# Autodesk Inventor assembly: Intake Full Assembly
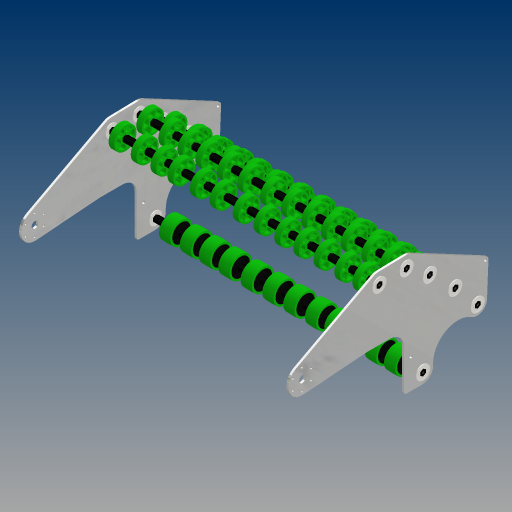
[picture p0: Inventor's stored thumbnail of the model, 512x512]
Saved by Autodesk Inventor 2024.3 (Build 283343000, 343)
## iProperties
Created: 2024-07-29
Part Number: Intake Full Assembly
Document SubType Name: Assembly
Designer: Kenji
Author: Kenji
## Documents named in this file (6)
- C:\Users\Kenji\Documents\GitHub\1622-2024-Summer-CAD-A-Thon\Intake\Intake Full Assembly.iam
- C:\Users\Kenji\Documents\GitHub\1622-2024-Summer-CAD-A-Thon\Intake\Intake Roller Plate.ipt
- C:\Users\Kenji\Documents\GitHub\1622-2024-Summer-CAD-A-Thon\COTS Library\Motion\Bearings\COTS_WCP-0783_1.125ODHexBearing.ipt
- C:\Users\Kenji\Documents\GitHub\1622-2024-Summer-CAD-A-Thon\Intake\Intake HexShaft 1.ipt
- C:\Users\Kenji\Documents\GitHub\1622-2024-Summer-CAD-A-Thon\Intake\am-3462 2IN Molded 500Hex Compliant Wheel REV2.ipt
- C:\Users\Kenji\Documents\GitHub\1622-2024-Summer-CAD-A-Thon\Intake\am-3155 2IN 500Hex Stealth Wheel REV2.iam
## Components (97 placed, 5 different names)
1. Intake Roller Plate:1 — Mate:13, Mate:14, Mate:15, Mate:16, Mate:17, Mate:18, Mate:19, Mate:20, Mate:21, Mate:22, Mate:23, Mate:24
2. Intake Roller Plate:2 — Mate:1, Mate:2, Mate:3, Mate:4, Mate:5, Mate:6, Mate:7, Mate:8, Mate:9, Mate:10, Mate:11, Mate:12
3. COTS_WCP-0783_1.125ODHexBearing:1 — Mate:5, Mate:7, Mate:25, Mate:32, Flush:11
4. COTS_WCP-0783_1.125ODHexBearing:2 — Mate:6, Mate:8, Mate:26, Mate:27, Flush:1
5. COTS_WCP-0783_1.125ODHexBearing:3 — Mate:4, Mate:11, Mate:31, Flush:9
6. COTS_WCP-0783_1.125ODHexBearing:4 — Mate:3, Mate:10, Flush:8
7. COTS_WCP-0783_1.125ODHexBearing:5 — Mate:1, Mate:9, Flush:4
8. COTS_WCP-0783_1.125ODHexBearing:6 — Mate:2, Mate:12, Flush:6
9. COTS_WCP-0783_1.125ODHexBearing:7 — Mate:17, Mate:24, Flush:10
10. COTS_WCP-0783_1.125ODHexBearing:8 — Mate:16, Mate:22, Mate:30, Flush:7
11. COTS_WCP-0783_1.125ODHexBearing:9 — Mate:15, Mate:21, Mate:29, Flush:5
12. COTS_WCP-0783_1.125ODHexBearing:10 — Mate:18, Mate:23, Mate:25, Flush:12
13. COTS_WCP-0783_1.125ODHexBearing:11 — Mate:13, Mate:19, Mate:26, Flush:2
14. COTS_WCP-0783_1.125ODHexBearing:12 — Mate:14, Mate:20, Mate:28, Flush:3, Mate:33, Mate:36, Mate:37, Mate:38, Mate:39, Mate:40
15. Intake HexShaft 1:1 — Mate:31, Flush:9, Flush:10, Mate:73, Mate:74, Mate:75, Mate:76, Mate:77, Mate:78, Mate:79, Mate:80, Mate:81, Mate:82, Mate:83, Mate:84, Mate:85
16. Intake HexShaft 1:2 — Mate:32, Flush:11, Flush:12, Mate:86, Mate:87, Mate:88, Mate:89, Mate:90, Mate:91, Mate:92, Mate:93, Mate:94, Mate:95, Mate:96, Mate:97, Mate:98
17. Intake HexShaft 1:3 — Mate:30, Flush:7, Flush:8, Mate:60, Mate:61, Mate:62, Mate:63, Mate:64, Mate:65, Mate:66, Mate:67, Mate:68, Mate:69, Mate:70, Mate:71, Mate:72
18. Intake HexShaft 1:4 — Mate:29, Flush:5, Flush:6, Mate:47, Mate:48, Mate:49, Mate:50, Mate:51, Mate:52, Mate:53, Mate:54, Mate:55, Mate:56, Mate:57, Mate:58, Mate:59
19. Intake HexShaft 1:5 — Mate:28, Flush:3, Flush:4, Mate:34, Mate:35, Mate:41, Mate:42, Mate:43, Mate:44, Mate:45
20. Intake HexShaft 1:6 — Mate:27, Flush:1, Flush:2, Mate:99, Mate:100, Mate:101, Mate:102, Mate:103, Mate:104, Mate:105, Mate:106, Mate:107, Mate:108, Mate:109, Mate:110
21. am-3462 2IN Molded 500Hex Compliant Wheel REV2:1 — Mate:45
22. am-3462 2IN Molded 500Hex Compliant Wheel REV2:2 — Mate:50
23. am-3462 2IN Molded 500Hex Compliant Wheel REV2:3 — Mate:51
24. am-3462 2IN Molded 500Hex Compliant Wheel REV2:4 — Mate:44
25. am-3462 2IN Molded 500Hex Compliant Wheel REV2:5 — Mate:40
26. am-3462 2IN Molded 500Hex Compliant Wheel REV2:6 — Mate:39
27. am-3462 2IN Molded 500Hex Compliant Wheel REV2:7 — Mate:42
28. am-3462 2IN Molded 500Hex Compliant Wheel REV2:8 — Mate:48
29. am-3462 2IN Molded 500Hex Compliant Wheel REV2:9 — Mate:52
30. am-3462 2IN Molded 500Hex Compliant Wheel REV2:10 — Mate:56
31. am-3462 2IN Molded 500Hex Compliant Wheel REV2:11 — Mate:55
32. am-3462 2IN Molded 500Hex Compliant Wheel REV2:12 — Mate:54
33. am-3462 2IN Molded 500Hex Compliant Wheel REV2:13 — Mate:53
34. am-3462 2IN Molded 500Hex Compliant Wheel REV2:14 — Mate:43
35. am-3462 2IN Molded 500Hex Compliant Wheel REV2:15 — Mate:41
36. am-3462 2IN Molded 500Hex Compliant Wheel REV2:16 — Mate:35
37. am-3462 2IN Molded 500Hex Compliant Wheel REV2:17 — Mate:37
38. am-3462 2IN Molded 500Hex Compliant Wheel REV2:19 — Mate:49
39. am-3462 2IN Molded 500Hex Compliant Wheel REV2:20 — Mate:47
40. am-3462 2IN Molded 500Hex Compliant Wheel REV2:21 — Mate:38
41. am-3462 2IN Molded 500Hex Compliant Wheel REV2:22 — Mate:36
42. am-3462 2IN Molded 500Hex Compliant Wheel REV2:23 — Mate:34
43. am-3462 2IN Molded 500Hex Compliant Wheel REV2:24 — Mate:33
44. am-3462 2IN Molded 500Hex Compliant Wheel REV2:25 — Mate:59
45. am-3462 2IN Molded 500Hex Compliant Wheel REV2:26 — Mate:58
46. am-3462 2IN Molded 500Hex Compliant Wheel REV2:27 — Mate:57
47. am-3462 2IN Molded 500Hex Compliant Wheel REV2:28 — Mate:65
48. am-3462 2IN Molded 500Hex Compliant Wheel REV2:29 — Mate:66
49. am-3462 2IN Molded 500Hex Compliant Wheel REV2:30 — Mate:67
50. am-3462 2IN Molded 500Hex Compliant Wheel REV2:31 — Mate:63
51. am-3462 2IN Molded 500Hex Compliant Wheel REV2:32 — Mate:68
52. am-3462 2IN Molded 500Hex Compliant Wheel REV2:33 — Mate:61
53. am-3462 2IN Molded 500Hex Compliant Wheel REV2:34 — Mate:60
54. am-3462 2IN Molded 500Hex Compliant Wheel REV2:35 — Mate:62
55. am-3462 2IN Molded 500Hex Compliant Wheel REV2:36 — Mate:64
56. am-3462 2IN Molded 500Hex Compliant Wheel REV2:37 — Mate:71
57. am-3462 2IN Molded 500Hex Compliant Wheel REV2:38 — Mate:70
58. am-3462 2IN Molded 500Hex Compliant Wheel REV2:39 — Mate:69
59. am-3462 2IN Molded 500Hex Compliant Wheel REV2:40 — Mate:72
60. am-3462 2IN Molded 500Hex Compliant Wheel REV2:41 — Mate:73
61. am-3462 2IN Molded 500Hex Compliant Wheel REV2:42 — Mate:75
62. am-3462 2IN Molded 500Hex Compliant Wheel REV2:43 — Mate:74
63. am-3462 2IN Molded 500Hex Compliant Wheel REV2:44 — Mate:76
64. am-3462 2IN Molded 500Hex Compliant Wheel REV2:45 — Mate:78
65. am-3462 2IN Molded 500Hex Compliant Wheel REV2:46 — Mate:77
66. am-3462 2IN Molded 500Hex Compliant Wheel REV2:47 — Mate:79
67. am-3462 2IN Molded 500Hex Compliant Wheel REV2:48 — Mate:80
68. am-3462 2IN Molded 500Hex Compliant Wheel REV2:49 — Mate:81
69. am-3462 2IN Molded 500Hex Compliant Wheel REV2:50 — Mate:84
70. am-3462 2IN Molded 500Hex Compliant Wheel REV2:51 — Mate:83
71. am-3462 2IN Molded 500Hex Compliant Wheel REV2:52 — Mate:82
72. am-3462 2IN Molded 500Hex Compliant Wheel REV2:53 — Mate:85
73. am-3462 2IN Molded 500Hex Compliant Wheel REV2:54 — Mate:86
74. am-3462 2IN Molded 500Hex Compliant Wheel REV2:55 — Mate:87
75. am-3462 2IN Molded 500Hex Compliant Wheel REV2:56 — Mate:88
76. am-3462 2IN Molded 500Hex Compliant Wheel REV2:57 — Mate:91
77. am-3462 2IN Molded 500Hex Compliant Wheel REV2:58 — Mate:90
78. am-3462 2IN Molded 500Hex Compliant Wheel REV2:59 — Mate:89
79. am-3462 2IN Molded 500Hex Compliant Wheel REV2:60 — Mate:92
80. am-3462 2IN Molded 500Hex Compliant Wheel REV2:61 — Mate:93
81. am-3462 2IN Molded 500Hex Compliant Wheel REV2:62 — Mate:94
82. am-3462 2IN Molded 500Hex Compliant Wheel REV2:63 — Mate:95
83. am-3462 2IN Molded 500Hex Compliant Wheel REV2:64 — Mate:96
84. am-3462 2IN Molded 500Hex Compliant Wheel REV2:65 — Mate:97
85. am-3462 2IN Molded 500Hex Compliant Wheel REV2:66 — Mate:98
86. am-3155 2IN 500Hex Stealth Wheel REV2:1 [sub-assembly] — Mate:99
87. am-3155 2IN 500Hex Stealth Wheel REV2:2 [sub-assembly] — Mate:100
88. am-3155 2IN 500Hex Stealth Wheel REV2:3 [sub-assembly] — Mate:101
89. am-3155 2IN 500Hex Stealth Wheel REV2:4 [sub-assembly] — Mate:102
90. am-3155 2IN 500Hex Stealth Wheel REV2:5 [sub-assembly] — Mate:103
91. am-3155 2IN 500Hex Stealth Wheel REV2:6 [sub-assembly] — Mate:104
92. am-3155 2IN 500Hex Stealth Wheel REV2:7 [sub-assembly] — Mate:105
93. am-3155 2IN 500Hex Stealth Wheel REV2:8 [sub-assembly] — Mate:106
94. am-3155 2IN 500Hex Stealth Wheel REV2:9 [sub-assembly] — Mate:108
95. am-3155 2IN 500Hex Stealth Wheel REV2:10 [sub-assembly] — Mate:109
96. am-3155 2IN 500Hex Stealth Wheel REV2:11 [sub-assembly] — Mate:110
97. am-3155 2IN 500Hex Stealth Wheel REV2:13 [sub-assembly] — Mate:107
## Relationships (121: Mate 109, Flush 12)
- Mate:1: Intake Roller Plate:2 ↔ COTS_WCP-0783_1.125ODHexBearing:5
- Mate:2: Intake Roller Plate:2 ↔ COTS_WCP-0783_1.125ODHexBearing:6
- Mate:3: Intake Roller Plate:2 ↔ COTS_WCP-0783_1.125ODHexBearing:4
- Mate:4: Intake Roller Plate:2 ↔ COTS_WCP-0783_1.125ODHexBearing:3
- Mate:5: Intake Roller Plate:2 ↔ COTS_WCP-0783_1.125ODHexBearing:1
- Mate:6: Intake Roller Plate:2 ↔ COTS_WCP-0783_1.125ODHexBearing:2
- Mate:7: Intake Roller Plate:2 ↔ COTS_WCP-0783_1.125ODHexBearing:1
- Mate:8: Intake Roller Plate:2 ↔ COTS_WCP-0783_1.125ODHexBearing:2
- Mate:9: Intake Roller Plate:2 ↔ COTS_WCP-0783_1.125ODHexBearing:5
- Mate:10: Intake Roller Plate:2 ↔ COTS_WCP-0783_1.125ODHexBearing:4
- Mate:11: Intake Roller Plate:2 ↔ COTS_WCP-0783_1.125ODHexBearing:3
- Mate:12: Intake Roller Plate:2 ↔ COTS_WCP-0783_1.125ODHexBearing:6
- Mate:13: Intake Roller Plate:1 ↔ COTS_WCP-0783_1.125ODHexBearing:11
- Mate:14: Intake Roller Plate:1 ↔ COTS_WCP-0783_1.125ODHexBearing:12
- Mate:15: Intake Roller Plate:1 ↔ COTS_WCP-0783_1.125ODHexBearing:9
- Mate:16: Intake Roller Plate:1 ↔ COTS_WCP-0783_1.125ODHexBearing:8
- Mate:17: Intake Roller Plate:1 ↔ COTS_WCP-0783_1.125ODHexBearing:7
- Mate:18: Intake Roller Plate:1 ↔ COTS_WCP-0783_1.125ODHexBearing:10
- Mate:19: Intake Roller Plate:1 ↔ COTS_WCP-0783_1.125ODHexBearing:11
- Mate:20: Intake Roller Plate:1 ↔ COTS_WCP-0783_1.125ODHexBearing:12
- Mate:21: Intake Roller Plate:1 ↔ COTS_WCP-0783_1.125ODHexBearing:9
- Mate:22: Intake Roller Plate:1 ↔ COTS_WCP-0783_1.125ODHexBearing:8
- Mate:23: Intake Roller Plate:1 ↔ COTS_WCP-0783_1.125ODHexBearing:10
- Mate:24: Intake Roller Plate:1 ↔ COTS_WCP-0783_1.125ODHexBearing:7
- Mate:25: COTS_WCP-0783_1.125ODHexBearing:1 ↔ COTS_WCP-0783_1.125ODHexBearing:10
- Mate:26: COTS_WCP-0783_1.125ODHexBearing:2 ↔ COTS_WCP-0783_1.125ODHexBearing:11
- Mate:27: COTS_WCP-0783_1.125ODHexBearing:2 ↔ Intake HexShaft 1:6
- Flush:1: COTS_WCP-0783_1.125ODHexBearing:2 ↔ Intake HexShaft 1:6
- Flush:2: COTS_WCP-0783_1.125ODHexBearing:11 ↔ Intake HexShaft 1:6
- Mate:28: COTS_WCP-0783_1.125ODHexBearing:12 ↔ Intake HexShaft 1:5
- Flush:3: COTS_WCP-0783_1.125ODHexBearing:12 ↔ Intake HexShaft 1:5
- Flush:4: COTS_WCP-0783_1.125ODHexBearing:5 ↔ Intake HexShaft 1:5
- Mate:29: COTS_WCP-0783_1.125ODHexBearing:9 ↔ Intake HexShaft 1:4
- Flush:5: COTS_WCP-0783_1.125ODHexBearing:9 ↔ Intake HexShaft 1:4
- Flush:6: COTS_WCP-0783_1.125ODHexBearing:6 ↔ Intake HexShaft 1:4
- Mate:30: COTS_WCP-0783_1.125ODHexBearing:8 ↔ Intake HexShaft 1:3
- Flush:7: COTS_WCP-0783_1.125ODHexBearing:8 ↔ Intake HexShaft 1:3
- Flush:8: COTS_WCP-0783_1.125ODHexBearing:4 ↔ Intake HexShaft 1:3
- Mate:31: COTS_WCP-0783_1.125ODHexBearing:3 ↔ Intake HexShaft 1:1
- Flush:9: COTS_WCP-0783_1.125ODHexBearing:3 ↔ Intake HexShaft 1:1
- Flush:10: COTS_WCP-0783_1.125ODHexBearing:7 ↔ Intake HexShaft 1:1
- Mate:32: COTS_WCP-0783_1.125ODHexBearing:1 ↔ Intake HexShaft 1:2
- Flush:11: COTS_WCP-0783_1.125ODHexBearing:1 ↔ Intake HexShaft 1:2
- Flush:12: COTS_WCP-0783_1.125ODHexBearing:10 ↔ Intake HexShaft 1:2
- Mate:33: COTS_WCP-0783_1.125ODHexBearing:12 ↔ am-3462 2IN Molded 500Hex Compliant Wheel REV2:24
- Mate:34: Intake HexShaft 1:5 ↔ am-3462 2IN Molded 500Hex Compliant Wheel REV2:23
- Mate:35: Intake HexShaft 1:5 ↔ am-3462 2IN Molded 500Hex Compliant Wheel REV2:16
- Mate:36: COTS_WCP-0783_1.125ODHexBearing:12 ↔ am-3462 2IN Molded 500Hex Compliant Wheel REV2:22
- Mate:37: COTS_WCP-0783_1.125ODHexBearing:12 ↔ am-3462 2IN Molded 500Hex Compliant Wheel REV2:17
- Mate:38: COTS_WCP-0783_1.125ODHexBearing:12 ↔ am-3462 2IN Molded 500Hex Compliant Wheel REV2:21
- Mate:39: COTS_WCP-0783_1.125ODHexBearing:12 ↔ am-3462 2IN Molded 500Hex Compliant Wheel REV2:6
- Mate:40: COTS_WCP-0783_1.125ODHexBearing:12 ↔ am-3462 2IN Molded 500Hex Compliant Wheel REV2:5
- Mate:41: Intake HexShaft 1:5 ↔ am-3462 2IN Molded 500Hex Compliant Wheel REV2:15
- Mate:42: Intake HexShaft 1:5 ↔ am-3462 2IN Molded 500Hex Compliant Wheel REV2:7
- Mate:43: Intake HexShaft 1:5 ↔ am-3462 2IN Molded 500Hex Compliant Wheel REV2:14
- Mate:44: Intake HexShaft 1:5 ↔ am-3462 2IN Molded 500Hex Compliant Wheel REV2:4
- Mate:45: Intake HexShaft 1:5 ↔ am-3462 2IN Molded 500Hex Compliant Wheel REV2:1
- Mate:47: Intake HexShaft 1:4 ↔ am-3462 2IN Molded 500Hex Compliant Wheel REV2:20
- Mate:48: Intake HexShaft 1:4 ↔ am-3462 2IN Molded 500Hex Compliant Wheel REV2:8
- Mate:49: Intake HexShaft 1:4 ↔ am-3462 2IN Molded 500Hex Compliant Wheel REV2:19
- Mate:50: Intake HexShaft 1:4 ↔ am-3462 2IN Molded 500Hex Compliant Wheel REV2:2
- Mate:51: Intake HexShaft 1:4 ↔ am-3462 2IN Molded 500Hex Compliant Wheel REV2:3
- Mate:52: Intake HexShaft 1:4 ↔ am-3462 2IN Molded 500Hex Compliant Wheel REV2:9
- Mate:53: Intake HexShaft 1:4 ↔ am-3462 2IN Molded 500Hex Compliant Wheel REV2:13
- Mate:54: Intake HexShaft 1:4 ↔ am-3462 2IN Molded 500Hex Compliant Wheel REV2:12
- Mate:55: Intake HexShaft 1:4 ↔ am-3462 2IN Molded 500Hex Compliant Wheel REV2:11
- Mate:56: Intake HexShaft 1:4 ↔ am-3462 2IN Molded 500Hex Compliant Wheel REV2:10
- Mate:57: Intake HexShaft 1:4 ↔ am-3462 2IN Molded 500Hex Compliant Wheel REV2:27
- Mate:58: Intake HexShaft 1:4 ↔ am-3462 2IN Molded 500Hex Compliant Wheel REV2:26
- Mate:59: Intake HexShaft 1:4 ↔ am-3462 2IN Molded 500Hex Compliant Wheel REV2:25
- Mate:60: Intake HexShaft 1:3 ↔ am-3462 2IN Molded 500Hex Compliant Wheel REV2:34
- Mate:61: Intake HexShaft 1:3 ↔ am-3462 2IN Molded 500Hex Compliant Wheel REV2:33
- Mate:62: Intake HexShaft 1:3 ↔ am-3462 2IN Molded 500Hex Compliant Wheel REV2:35
- Mate:63: Intake HexShaft 1:3 ↔ am-3462 2IN Molded 500Hex Compliant Wheel REV2:31
- Mate:64: Intake HexShaft 1:3 ↔ am-3462 2IN Molded 500Hex Compliant Wheel REV2:36
- Mate:65: Intake HexShaft 1:3 ↔ am-3462 2IN Molded 500Hex Compliant Wheel REV2:28
- Mate:66: Intake HexShaft 1:3 ↔ am-3462 2IN Molded 500Hex Compliant Wheel REV2:29
- Mate:67: Intake HexShaft 1:3 ↔ am-3462 2IN Molded 500Hex Compliant Wheel REV2:30
- Mate:68: Intake HexShaft 1:3 ↔ am-3462 2IN Molded 500Hex Compliant Wheel REV2:32
- Mate:69: Intake HexShaft 1:3 ↔ am-3462 2IN Molded 500Hex Compliant Wheel REV2:39
- Mate:70: Intake HexShaft 1:3 ↔ am-3462 2IN Molded 500Hex Compliant Wheel REV2:38
- Mate:71: Intake HexShaft 1:3 ↔ am-3462 2IN Molded 500Hex Compliant Wheel REV2:37
- Mate:72: Intake HexShaft 1:3 ↔ am-3462 2IN Molded 500Hex Compliant Wheel REV2:40
- Mate:73: Intake HexShaft 1:1 ↔ am-3462 2IN Molded 500Hex Compliant Wheel REV2:41
- Mate:74: Intake HexShaft 1:1 ↔ am-3462 2IN Molded 500Hex Compliant Wheel REV2:43
- Mate:75: Intake HexShaft 1:1 ↔ am-3462 2IN Molded 500Hex Compliant Wheel REV2:42
- Mate:76: Intake HexShaft 1:1 ↔ am-3462 2IN Molded 500Hex Compliant Wheel REV2:44
- Mate:77: Intake HexShaft 1:1 ↔ am-3462 2IN Molded 500Hex Compliant Wheel REV2:46
- Mate:78: Intake HexShaft 1:1 ↔ am-3462 2IN Molded 500Hex Compliant Wheel REV2:45
- Mate:79: Intake HexShaft 1:1 ↔ am-3462 2IN Molded 500Hex Compliant Wheel REV2:47
- Mate:80: Intake HexShaft 1:1 ↔ am-3462 2IN Molded 500Hex Compliant Wheel REV2:48
- Mate:81: Intake HexShaft 1:1 ↔ am-3462 2IN Molded 500Hex Compliant Wheel REV2:49
- Mate:82: Intake HexShaft 1:1 ↔ am-3462 2IN Molded 500Hex Compliant Wheel REV2:52
- Mate:83: Intake HexShaft 1:1 ↔ am-3462 2IN Molded 500Hex Compliant Wheel REV2:51
- Mate:84: Intake HexShaft 1:1 ↔ am-3462 2IN Molded 500Hex Compliant Wheel REV2:50
- Mate:85: Intake HexShaft 1:1 ↔ am-3462 2IN Molded 500Hex Compliant Wheel REV2:53
- Mate:86: Intake HexShaft 1:2 ↔ am-3462 2IN Molded 500Hex Compliant Wheel REV2:54
- Mate:87: Intake HexShaft 1:2 ↔ am-3462 2IN Molded 500Hex Compliant Wheel REV2:55
- Mate:88: Intake HexShaft 1:2 ↔ am-3462 2IN Molded 500Hex Compliant Wheel REV2:56
- Mate:89: Intake HexShaft 1:2 ↔ am-3462 2IN Molded 500Hex Compliant Wheel REV2:59
- Mate:90: Intake HexShaft 1:2 ↔ am-3462 2IN Molded 500Hex Compliant Wheel REV2:58
- Mate:91: Intake HexShaft 1:2 ↔ am-3462 2IN Molded 500Hex Compliant Wheel REV2:57
- Mate:92: Intake HexShaft 1:2 ↔ am-3462 2IN Molded 500Hex Compliant Wheel REV2:60
- Mate:93: Intake HexShaft 1:2 ↔ am-3462 2IN Molded 500Hex Compliant Wheel REV2:61
- Mate:94: Intake HexShaft 1:2 ↔ am-3462 2IN Molded 500Hex Compliant Wheel REV2:62
- Mate:95: Intake HexShaft 1:2 ↔ am-3462 2IN Molded 500Hex Compliant Wheel REV2:63
- Mate:96: Intake HexShaft 1:2 ↔ am-3462 2IN Molded 500Hex Compliant Wheel REV2:64
- Mate:97: Intake HexShaft 1:2 ↔ am-3462 2IN Molded 500Hex Compliant Wheel REV2:65
- Mate:98: Intake HexShaft 1:2 ↔ am-3462 2IN Molded 500Hex Compliant Wheel REV2:66
- Mate:99: Intake HexShaft 1:6 ↔ am-3155 2IN 500Hex Stealth Wheel REV2:1
- Mate:100: Intake HexShaft 1:6 ↔ am-3155 2IN 500Hex Stealth Wheel REV2:2
- Mate:101: Intake HexShaft 1:6 ↔ am-3155 2IN 500Hex Stealth Wheel REV2:3
- Mate:102: Intake HexShaft 1:6 ↔ am-3155 2IN 500Hex Stealth Wheel REV2:4
- Mate:103: Intake HexShaft 1:6 ↔ am-3155 2IN 500Hex Stealth Wheel REV2:5
- Mate:104: Intake HexShaft 1:6 ↔ am-3155 2IN 500Hex Stealth Wheel REV2:6
- Mate:105: Intake HexShaft 1:6 ↔ am-3155 2IN 500Hex Stealth Wheel REV2:7
- Mate:106: Intake HexShaft 1:6 ↔ am-3155 2IN 500Hex Stealth Wheel REV2:8
- Mate:107: Intake HexShaft 1:6 ↔ am-3155 2IN 500Hex Stealth Wheel REV2:13
- Mate:108: Intake HexShaft 1:6 ↔ am-3155 2IN 500Hex Stealth Wheel REV2:9
- Mate:109: Intake HexShaft 1:6 ↔ am-3155 2IN 500Hex Stealth Wheel REV2:10
- Mate:110: Intake HexShaft 1:6 ↔ am-3155 2IN 500Hex Stealth Wheel REV2:11
